# Autodesk Inventor assembly: dsbc-32-100-ppva-n3-3d-model-1-en
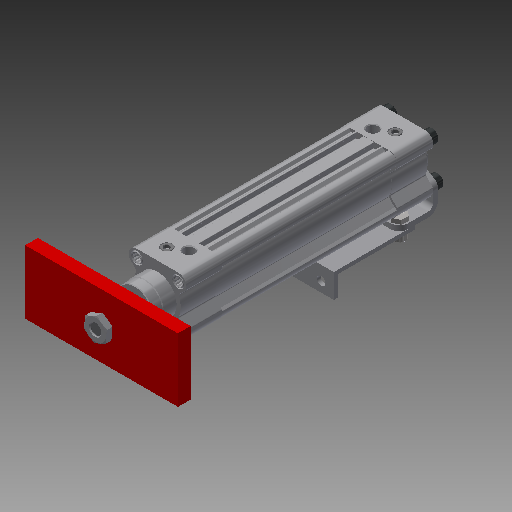
[picture p0: Inventor's stored thumbnail of the model, 512x512]
Saved by Autodesk Inventor 2019 (Build 230136000, 136)
## iProperties
Created: 2016-05-18
Part Number: dsbc-32-100-ppva-n3-3d-model-1-en
Description: STEP AP214
Document SubType Name: Assembly
Designer: felix
Mass: 334.574 g
Surface Area: 1178.13 cm^2
Volume: 321.299 cm^3
Density: 1.04132 g/cm^3
Sending System: PARTsolutions
Title: C:/Users/jhr/Documents/Festo/CADBasket/Export/step 2.14/d/dsbc/1376426 DSBC-32-100-PPVA-N3---(0).stp
Revision Number: NONE
## Documents named in this file (7)
- D:\Downloads\dsbc-32-100-ppva-n3-3d-model-1-en.iam
- D:\Downloads\HI_1463250 DSBC-32-100-PPVA_(Z).ipt
- D:\Downloads\HI_1463250 DSBC-32-100_(K).ipt
- D:\Downloads\_DIN-439-B - M10x1.25(F).ipt
- D:\Documents\Inventor\Content Center Files\Empuje.ipt
- D:\Downloads\hnc-32-3d-model-1-en.iam
- D:\Downloads\_DIN-912 - M6x18(F).ipt
## Components (10 placed, 7 different names)
1. NAUO1 — Mate:1, Flush:1, Mate:7, Mate:8, Mate:9, Mate:11, Mate:12, Mate:14, Mate:17
2. NAUO2 — Mate:1, Flush:1, Mate:2, Mate:3, Flush:2, Mate:5
3. NAUO3 — Mate:2, Mate:4
4. Empuje:1 — Mate:3, Flush:2, Mate:4, Mate:6
5. _DIN-439-B - M10x1.25(F):2 — Mate:5, Mate:6
6. hnc-32-3d-model-1-en:1 [sub-assembly] — Mate:7, Mate:8, Mate:9, Mate:10, Mate:13, Mate:15, Mate:16
7. _DIN-912 - M6x18(F):1 — Mate:11, Mate:17
8. _DIN-912 - M6x18(F):2 — Mate:10, Mate:16
9. _DIN-912 - M6x18(F):3 — Mate:12, Mate:14
10. _DIN-912 - M6x18(F):4 — Mate:13, Mate:15
## Relationships (19: Mate 17, Flush 2)
- Mate:1: NAUO1 ↔ NAUO2
- Flush:1 (30 mm): NAUO1 ↔ NAUO2
- Mate:2: NAUO2 ↔ NAUO3
- Mate:3: NAUO2 ↔ Empuje:1
- Flush:2 (-4 mm): NAUO2 ↔ Empuje:1
- Mate:4: NAUO3 ↔ Empuje:1
- Mate:5: NAUO2 ↔ _DIN-439-B - M10x1.25(F):2
- Mate:6: Empuje:1 ↔ _DIN-439-B - M10x1.25(F):2
- Mate:7: NAUO1 ↔ hnc-32-3d-model-1-en:1
- Mate:8: NAUO1 ↔ hnc-32-3d-model-1-en:1
- Mate:9: NAUO1 ↔ hnc-32-3d-model-1-en:1
- Mate:10: hnc-32-3d-model-1-en:1 ↔ _DIN-912 - M6x18(F):2
- Mate:11: NAUO1 ↔ _DIN-912 - M6x18(F):1
- Mate:12: NAUO1 ↔ _DIN-912 - M6x18(F):3
- Mate:13: hnc-32-3d-model-1-en:1 ↔ _DIN-912 - M6x18(F):4
- Mate:14: NAUO1 ↔ _DIN-912 - M6x18(F):3
- Mate:15: hnc-32-3d-model-1-en:1 ↔ _DIN-912 - M6x18(F):4
- Mate:16: hnc-32-3d-model-1-en:1 ↔ _DIN-912 - M6x18(F):2
- Mate:17: NAUO1 ↔ _DIN-912 - M6x18(F):1
